# Autodesk Inventor assembly: TorsoPelvisUnit
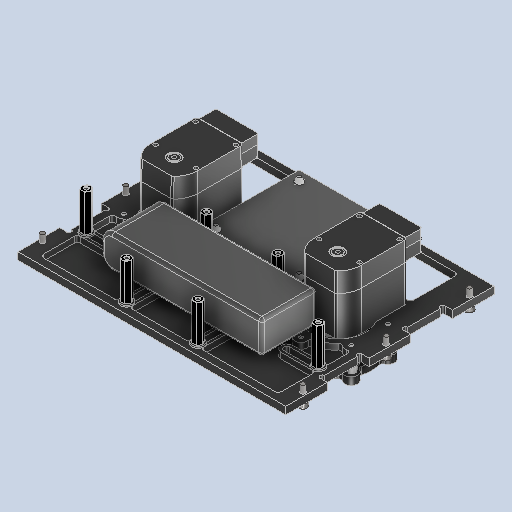
[picture p0: Inventor's stored thumbnail of the model, 512x512]
Saved by Autodesk Inventor 2024.2 (Build 282272000, 272)
## iProperties
Created: 2024-01-05
Part Number: TorsoPelvisUnit
Document SubType Name: Assembly
Designer: Masato Kubotera
Mass: 796.863 g
Surface Area: 1429.36 cm^2
Volume: 306.795 cm^3
Density: 2.59738 g/cm^3
Author: Masato Kubotera
## Documents named in this file (12)
- C:\Users\masato\OneDrive - Chiba Institute of Technology\CIT Brains\RoboCup2024\Mechanic\SUSTAINA-OP2-DEV\NativeFiles\Boby\Torso\TorsoPelvis\TorsoPelvisUnit.iam
- C:\Users\masato\OneDrive - Chiba Institute of Technology\CIT Brains\RoboCup2024\Mechanic\SUSTAINA-OP2-DEV\NativeFiles\Boby\Torso\TorsoPelvis\TorsoPelvisLowerFrame.ipt
- C:\Users\masato\OneDrive - Chiba Institute of Technology\CIT Brains\RoboCup2024\Mechanic\SUSTAINA-OP2-DEV\NativeFiles\Boby\CommonDesignedComponents\CrossRollerBearingUnit\CrossRollerBearingUnit.iam
- C:\Users\masato\OneDrive - Chiba Institute of Technology\CIT Brains\RoboCup2024\Mechanic\SUSTAINA-OP2-DEV\NativeFiles\Boby\COTS\Screws\CapScrew\UC-0310.ipt
- C:\Users\masato\OneDrive - Chiba Institute of Technology\CIT Brains\RoboCup2024\Mechanic\SUSTAINA-OP2-DEV\NativeFiles\Boby\COTS\Screws\CapScrew\FC-2615EB.ipt
- C:\Users\masato\OneDrive - Chiba Institute of Technology\CIT Brains\RoboCup2024\Mechanic\SUSTAINA-OP2-DEV\NativeFiles\Boby\COTS\Spacers\WBN-305.ipt
- C:\Users\masato\OneDrive - Chiba Institute of Technology\CIT Brains\RoboCup2024\Mechanic\SUSTAINA-OP2-DEV\NativeFiles\Boby\CustomElectronicComponents\SUSTAINA-POWER-INPUT-BORAD.ipt
- C:\Users\masato\OneDrive - Chiba Institute of Technology\CIT Brains\RoboCup2024\Mechanic\SUSTAINA-OP2-DEV\NativeFiles\Boby\COTS\Actuators\PMX-SCR-9203HV.ipt
- C:\Users\masato\OneDrive - Chiba Institute of Technology\CIT Brains\RoboCup2024\Mechanic\SUSTAINA-OP2-DEV\NativeFiles\Boby\COTS\ElectronicComponents\Batteries\Lipo-3250-3S-Pack-3.ipt
- C:\Users\masato\OneDrive - Chiba Institute of Technology\CIT Brains\RoboCup2024\Mechanic\SUSTAINA-OP2-DEV\NativeFiles\Boby\COTS\ElectronicComponents\Batteries\Lipo-2800-3S-Pack-3.ipt
- C:\Users\masato\OneDrive - Chiba Institute of Technology\CIT Brains\RoboCup2024\Mechanic\SUSTAINA-OP2-DEV\NativeFiles\Boby\COTS\Bushes\L3040-8110TB.ipt
- C:\Users\masato\OneDrive - Chiba Institute of Technology\CIT Brains\RoboCup2024\Mechanic\SUSTAINA-OP2-DEV\NativeFiles\Boby\COTS\Spacers\BSL-325BE.ipt
## Components (46 placed, 11 different names)
1. CrossRollerBearingUnit:1 [sub-assembly] — Insert:1, Insert:2
2. CrossRollerBearingUnit:2 [sub-assembly] — Insert:42, Insert:43
3. Lipo-2800-3S-Pack-3:1
4. L3040-8110TB:1 — Insert:85, Insert:91, Insert:93
5. L3040-8110TB:2 — Insert:86, Insert:92, Insert:94
6. L3040-8110TB:3 — Insert:87, Insert:89, Insert:95
7. L3040-8110TB:4 — Insert:88, Insert:90, Insert:96
8. L3040-8110TB:5 — Insert:91, Insert:107
9. L3040-8110TB:6 — Insert:92, Insert:108
10. L3040-8110TB:7 — Insert:89, Insert:105
11. L3040-8110TB:8 — Insert:90, Insert:106
12. UC-0310:7 — Insert:85
13. UC-0310:8 — Insert:86
14. UC-0310:9 — Insert:87
15. UC-0310:10 — Insert:88
16. L3040-8110TB:9 — Insert:101
17. L3040-8110TB:10 — Insert:103
18. UC-0310:11
19. L3040-8110TB:11 — Insert:102
20. L3040-8110TB:12 — Insert:104
21. UC-0310:12
22. BSL-325BE:1 — Insert:103
23. BSL-325BE:2 — Insert:104
24. BSL-325BE:3 — Insert:105
25. BSL-325BE:4 — Insert:106
26. BSL-325BE:5 — Insert:107
27. BSL-325BE:6 — Insert:108
28. TorsoPelvisLowerFrame:1 — Flush:1, Flush:2, Flush:3, Insert:1, Insert:2, Insert:3, Insert:4, Insert:5, Insert:6, Insert:7, Insert:8, Insert:9, Insert:38, Insert:39, Insert:40, Insert:41, Insert:42, Insert:43, Insert:44, Insert:45, Insert:46, Insert:73, Insert:74, Insert:75, Insert:76, Insert:93, Insert:94, Insert:95, Insert:96, Insert:101, Insert:102
29. SUSTAINA-POWER-INPUT-BORAD:1 — Insert:81, Insert:82, Insert:83, Insert:84
30. PMX-SCR-9203HV:2 — Insert:3, Insert:4
31. PMX-SCR-9203HV:1 — Insert:38, Insert:39
32. Lipo-3250-3S-Pack-3:1
33. UC-0310:1 — Insert:5
34. UC-0310:2 — Insert:6
35. UC-0310:3 — Insert:7
36. UC-0310:4 — Insert:44
37. UC-0310:5 — Insert:45
38. UC-0310:6 — Insert:46
39. FC-2615EB:1 — Insert:8
40. FC-2615EB:2 — Insert:9
41. FC-2615EB:3 — Insert:40
42. FC-2615EB:4 — Insert:41
43. WBN-305:1 — Angle:1, Insert:73, Insert:81
44. WBN-305:2 — Angle:2, Insert:74, Insert:82
45. WBN-305:3 — Angle:3, Insert:75, Insert:83
46. WBN-305:4 — Angle:4, Insert:76, Insert:84
## Relationships (57: Insert 50, Angle 4, Flush 3)
- Flush:1: TorsoPelvisLowerFrame:1
- Flush:2: TorsoPelvisLowerFrame:1
- Flush:3: TorsoPelvisLowerFrame:1
- Insert:1: CrossRollerBearingUnit:1 ↔ TorsoPelvisLowerFrame:1
- Insert:2: CrossRollerBearingUnit:1 ↔ TorsoPelvisLowerFrame:1
- Insert:3: TorsoPelvisLowerFrame:1 ↔ PMX-SCR-9203HV:2
- Insert:4: TorsoPelvisLowerFrame:1 ↔ PMX-SCR-9203HV:2
- Insert:5: TorsoPelvisLowerFrame:1 ↔ UC-0310:1
- Insert:6: TorsoPelvisLowerFrame:1 ↔ UC-0310:2
- Insert:7: TorsoPelvisLowerFrame:1 ↔ UC-0310:3
- Insert:8: TorsoPelvisLowerFrame:1 ↔ FC-2615EB:1
- Insert:9: TorsoPelvisLowerFrame:1 ↔ FC-2615EB:2
- Insert:38: TorsoPelvisLowerFrame:1 ↔ PMX-SCR-9203HV:1
- Insert:39: TorsoPelvisLowerFrame:1 ↔ PMX-SCR-9203HV:1
- Insert:40: TorsoPelvisLowerFrame:1 ↔ FC-2615EB:3
- Insert:41: TorsoPelvisLowerFrame:1 ↔ FC-2615EB:4
- Insert:42: CrossRollerBearingUnit:2 ↔ TorsoPelvisLowerFrame:1
- Insert:43: CrossRollerBearingUnit:2 ↔ TorsoPelvisLowerFrame:1
- Insert:44: TorsoPelvisLowerFrame:1 ↔ UC-0310:4
- Insert:45: TorsoPelvisLowerFrame:1 ↔ UC-0310:5
- Insert:46: TorsoPelvisLowerFrame:1 ↔ UC-0310:6
- Angle:1 (0 deg): WBN-305:1
- Angle:2 (0 deg): WBN-305:2
- Angle:3 (0 deg): WBN-305:3
- Angle:4 (0 deg): WBN-305:4
- Insert:73: TorsoPelvisLowerFrame:1 ↔ WBN-305:1
- Insert:74: TorsoPelvisLowerFrame:1 ↔ WBN-305:2
- Insert:75: TorsoPelvisLowerFrame:1 ↔ WBN-305:3
- Insert:76: TorsoPelvisLowerFrame:1 ↔ WBN-305:4
- Insert:81: SUSTAINA-POWER-INPUT-BORAD:1 ↔ WBN-305:1
- Insert:82: SUSTAINA-POWER-INPUT-BORAD:1 ↔ WBN-305:2
- Insert:83: SUSTAINA-POWER-INPUT-BORAD:1 ↔ WBN-305:3
- Insert:84: SUSTAINA-POWER-INPUT-BORAD:1 ↔ WBN-305:4
- Insert:85: L3040-8110TB:1 ↔ UC-0310:7
- Insert:86: L3040-8110TB:2 ↔ UC-0310:8
- Insert:87: L3040-8110TB:3 ↔ UC-0310:9
- Insert:88: L3040-8110TB:4 ↔ UC-0310:10
- Insert:89 (5 mm): L3040-8110TB:3 ↔ L3040-8110TB:7
- Insert:90 (5 mm): L3040-8110TB:4 ↔ L3040-8110TB:8
- Insert:91 (5 mm): L3040-8110TB:1 ↔ L3040-8110TB:5
- Insert:92 (5 mm): L3040-8110TB:2 ↔ L3040-8110TB:6
- Insert:93: L3040-8110TB:1 ↔ TorsoPelvisLowerFrame:1
- Insert:94: L3040-8110TB:2 ↔ TorsoPelvisLowerFrame:1
- Insert:95: L3040-8110TB:3 ↔ TorsoPelvisLowerFrame:1
- Insert:96: L3040-8110TB:4 ↔ TorsoPelvisLowerFrame:1
- [Insert]: L3040-8110TB:9 ↔ UC-0310:11
- [Insert] (5 mm): L3040-8110TB:9 ↔ L3040-8110TB:10
- [Insert]: L3040-8110TB:11 ↔ UC-0310:12
- [Insert] (5 mm): L3040-8110TB:11 ↔ L3040-8110TB:12
- Insert:101: L3040-8110TB:9 ↔ TorsoPelvisLowerFrame:1
- Insert:102: L3040-8110TB:11 ↔ TorsoPelvisLowerFrame:1
- Insert:103: L3040-8110TB:10 ↔ BSL-325BE:1
- Insert:104: L3040-8110TB:12 ↔ BSL-325BE:2
- Insert:105: L3040-8110TB:7 ↔ BSL-325BE:3
- Insert:106: L3040-8110TB:8 ↔ BSL-325BE:4
- Insert:107: L3040-8110TB:5 ↔ BSL-325BE:5
- Insert:108: L3040-8110TB:6 ↔ BSL-325BE:6
## Named parameters: d111_d99 = 0 mm, d112_d105 = 5 mm, d113_d99 = 0 mm, d114_d105 = 5 mm
